# Autodesk Inventor assembly: 新型３クランクアセンブリ_MIR1
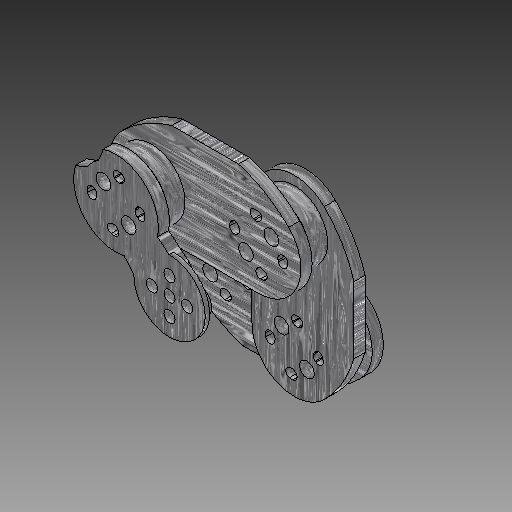
[picture p0: Inventor's stored thumbnail of the model, 512x512]
Saved by Autodesk Inventor 2019 (Build 230136000, 136)
## iProperties
Created: 2019-04-15
Part Number: 新型３クランクアセンブリ_MIR1
Material: 一般
Document SubType Name: Assembly
Designer: tanjihayato
Author: tanjihayato
## Documents named in this file (5)
- \\Mac\Home\Documents\Inventor\2019お遊び機体\新型３クランクアセンブリ_MIR1.iam
- \\Mac\Home\Documents\Inventor\2019お遊び機体\新型３クランク_MIR1.ipt
- \\Mac\Home\Documents\Inventor\2019お遊び機体\新型３脚カム_MIR.ipt
- \\Mac\Home\Documents\Inventor\2019お遊び機体\新型３クランク根本_MIR1.ipt
- \\Mac\Home\Documents\Inventor\2019お遊び機体\新型３涙_MIR1.ipt
## Components (9 placed, 4 different names)
1. 新型３クランク_MIR1:1 — メイト:1, 挿入:1, メイト:7, 挿入:7
2. 新型３クランク_MIR1:2 — メイト:2, 挿入:2, メイト:6, 挿入:6
3. 新型３クランク_MIR1:3 — メイト:3, 挿入:3, メイト:5, 挿入:5
4. 新型３脚カム_MIR:1 — メイト:1, 挿入:1, メイト:8, 挿入:8
5. 新型３脚カム_MIR:2 — メイト:7, 挿入:7, メイト:2, 挿入:2
6. 新型３脚カム_MIR:3 — メイト:6, 挿入:6, メイト:3, 挿入:3
7. 新型３脚カム_MIR:4 — メイト:5, 挿入:5, メイト:4, 挿入:4
8. 新型３クランク根本_MIR1:1 — メイト:4, 挿入:4
9. 新型３涙_MIR1:1 — メイト:8, 挿入:8
## Relationships (16: Mate 8, Insert 8)
- メイト:1 [Mate]: 新型３クランク_MIR1:1 ↔ 新型３脚カム_MIR:1
- 挿入:1 [Insert]: 新型３クランク_MIR1:1 ↔ 新型３脚カム_MIR:1
- メイト:7 [Mate]: 新型３クランク_MIR1:1 ↔ 新型３脚カム_MIR:2
- 挿入:7 [Insert]: 新型３クランク_MIR1:1 ↔ 新型３脚カム_MIR:2
- メイト:2 [Mate]: 新型３クランク_MIR1:2 ↔ 新型３脚カム_MIR:2
- 挿入:2 [Insert]: 新型３クランク_MIR1:2 ↔ 新型３脚カム_MIR:2
- メイト:6 [Mate]: 新型３クランク_MIR1:2 ↔ 新型３脚カム_MIR:3
- 挿入:6 [Insert]: 新型３クランク_MIR1:2 ↔ 新型３脚カム_MIR:3
- メイト:3 [Mate]: 新型３クランク_MIR1:3 ↔ 新型３脚カム_MIR:3
- 挿入:3 [Insert]: 新型３クランク_MIR1:3 ↔ 新型３脚カム_MIR:3
- メイト:5 [Mate]: 新型３クランク_MIR1:3 ↔ 新型３脚カム_MIR:4
- 挿入:5 [Insert]: 新型３クランク_MIR1:3 ↔ 新型３脚カム_MIR:4
- メイト:4 [Mate]: 新型３脚カム_MIR:4 ↔ 新型３クランク根本_MIR1:1
- 挿入:4 [Insert]: 新型３脚カム_MIR:4 ↔ 新型３クランク根本_MIR1:1
- メイト:8 [Mate]: 新型３脚カム_MIR:1 ↔ 新型３涙_MIR1:1
- 挿入:8 [Insert]: 新型３脚カム_MIR:1 ↔ 新型３涙_MIR1:1
